# Autodesk Inventor assembly: robot
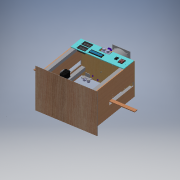
[picture p0: Inventor's stored thumbnail of the model, 180x180]
Saved by Autodesk Inventor 2017 (Build 210142000, 142)
## iProperties
Created: 2018-04-01
Part Number: robot
Document SubType Name: Assembly
Designer: franc
Mass: 1235.72 g
Surface Area: 6399.52 cm^2
Volume: 1204.8 cm^3
Density: 1.02566 g/cm^3
Author: franc
## Documents named in this file (16)
- C:\Users\franc\Desktop\EsialRobotik\Mecanique\2018\robot\robot.iam
- C:\Users\franc\Desktop\EsialRobotik\Mecanique\base_roulante\baseRoulante.iam
- C:\Users\franc\Desktop\EsialRobotik\Mecanique\2018\robot\socle-robot.ipt
- C:\Users\franc\Desktop\EsialRobotik\Mecanique\2018\robot\profile_alu.ipt
- C:\Users\franc\Desktop\EsialRobotik\Mecanique\2018\robot\abeille\lanceur-abeille.iam
- C:\Users\franc\Desktop\EsialRobotik\Mecanique\2018\robot\face-lateral.ipt
- C:\Users\franc\Desktop\EsialRobotik\Mecanique\2018\robot\abeille\lanceur-abeille 2.iam
- C:\Users\franc\Desktop\EsialRobotik\Mecanique\2018\robot\support_arriere.iam
- C:\Users\franc\Desktop\EsialRobotik\Mecanique\2018\robot\toit.ipt
- C:\Users\franc\Desktop\EsialRobotik\Mecanique\composants\SRF04\SRF04_sur_support.iam
- C:\Users\franc\Desktop\EsialRobotik\Mecanique\composants\Interrupteur\arret-urgence.ipt
- C:\Users\franc\Desktop\EsialRobotik\Mecanique\composants\RPlidar-A2M4\RPLIDAR A2.iam
- C:\Users\franc\Desktop\EsialRobotik\Mecanique\composants\Balises\support-balise.ipt
- C:\Users\franc\Desktop\EsialRobotik\Mecanique\composants\Balises\support-lidar.ipt
- C:\Users\franc\Desktop\EsialRobotik\Mecanique\composants\Balises\tige-filletee.ipt
- C:\Users\franc\Desktop\EsialRobotik\Mecanique\composants\Balises\cylindre-mat.ipt
## Components (26 placed, 15 different names)
1. baseRoulante:1 [sub-assembly] — Affleurement:1, Affleurement:2, Placage:1, Affleurement:6, Affleurement:7, Affleurement:9, Placage:29, Affleurement:10, Affleurement:12, Placage:32, Placage:34, Placage:66, Affleurement:31, Affleurement:32
2. socle-robot:1 — Affleurement:1, Affleurement:2, Placage:1, Placage:27, Affleurement:5, Affleurement:8, Placage:28, Placage:30, Affleurement:11, Placage:31, Placage:33, Affleurement:13, Placage:35, Placage:37, Affleurement:15, Placage:39
3. support_arriere:1 [sub-assembly] — Placage:43, Affleurement:16, Affleurement:17
4. arret-urgence:1 — Placage:53
5. SRF04_sur_support:1 [sub-assembly] — Placage:48, Affleurement:23, Placage:49
6. SRF04_sur_support:2 [sub-assembly] — Placage:45, Affleurement:20, Placage:52
7. SRF04_sur_support:3 [sub-assembly] — Placage:46, Affleurement:21, Placage:51
8. SRF04_sur_support:4 [sub-assembly] — Placage:47, Affleurement:22, Placage:50
9. toit:1 — Placage:44, Affleurement:18, Affleurement:19, Placage:45, Placage:46, Placage:47, Affleurement:20, Affleurement:21, Affleurement:22, Placage:48, Affleurement:23, Placage:49, Placage:50, Placage:51, Placage:52, Placage:53, Affleurement:24, Affleurement:25
10. lanceur-abeille 2:1 [sub-assembly] — Placage:40, Placage:41, Placage:42
11. lanceur-abeille:1 [sub-assembly] — Placage:36, Placage:37, Affleurement:14
12. profile_alu:1 — Affleurement:7, Affleurement:8, Placage:28, Placage:43
13. profile_alu:2 — Affleurement:9, Placage:29, Placage:30, Placage:38
14. profile_alu:3 — Affleurement:12, Placage:32, Placage:33
15. profile_alu:4 — Affleurement:10, Affleurement:11, Placage:31, Affleurement:17
16. face-lateral:1 — Placage:34, Affleurement:13, Placage:35, Placage:36, Affleurement:14, Affleurement:16, Placage:44, Affleurement:18, Affleurement:19
17. face-lateral:2 — Placage:38, Affleurement:15, Placage:39, Placage:40, Placage:41, Placage:42
18. cylindre-mat:1 — Placage:68, Tangente:1, Tangente:2
19. RPLIDAR A2:1 [sub-assembly] — Placage:54, Placage:55, Placage:56
20. support-balise:1 — Placage:61, Placage:62, Placage:63, Placage:68, Tangente:1, Tangente:2
21. support-lidar:1 — Placage:54, Placage:55, Placage:56, Placage:57, Placage:58, Placage:59, Placage:60, Placage:61, Placage:66, Affleurement:30, Placage:67
22. tige-filletee:1 — Placage:60, Placage:62, Affleurement:28
23. tige-filletee:2 — Placage:59, Affleurement:26, Placage:64
24. tige-filletee:3 — Placage:58, Placage:63, Affleurement:29
25. tige-filletee:4 — Placage:57, Placage:65, Affleurement:27
26. support-balise:2 — Affleurement:26, Placage:64, Placage:65, Affleurement:27, Affleurement:28, Affleurement:29, Affleurement:31
## Relationships (75: Mate 43, Flush 30, Tangent 2)
- Affleurement:1 [Flush] (5 mm): baseRoulante:1 ↔ socle-robot:1
- Affleurement:2 [Flush] (54 mm): baseRoulante:1 ↔ socle-robot:1
- Placage:1 [Mate]: baseRoulante:1 ↔ socle-robot:1
- Placage:27 [Mate]: socle-robot:1
- Affleurement:5 [Flush]: socle-robot:1
- Affleurement:6 [Flush] (340 mm): baseRoulante:1
- Affleurement:7 [Flush]: baseRoulante:1 ↔ profile_alu:1
- Affleurement:8 [Flush]: socle-robot:1 ↔ profile_alu:1
- Placage:28 [Mate]: socle-robot:1 ↔ profile_alu:1
- Affleurement:9 [Flush]: baseRoulante:1 ↔ profile_alu:2
- Placage:29 [Mate]: baseRoulante:1 ↔ profile_alu:2
- Placage:30 [Mate]: socle-robot:1 ↔ profile_alu:2
- Affleurement:10 [Flush]: baseRoulante:1 ↔ profile_alu:4
- Affleurement:11 [Flush]: socle-robot:1 ↔ profile_alu:4
- Placage:31 [Mate]: socle-robot:1 ↔ profile_alu:4
- Affleurement:12 [Flush]: baseRoulante:1 ↔ profile_alu:3
- Placage:32 [Mate]: baseRoulante:1 ↔ profile_alu:3
- Placage:33 [Mate]: socle-robot:1 ↔ profile_alu:3
- Placage:34 [Mate]: baseRoulante:1 ↔ face-lateral:1
- Affleurement:13 [Flush]: socle-robot:1 ↔ face-lateral:1
- Placage:35 [Mate]: socle-robot:1 ↔ face-lateral:1
- Placage:36 [Mate]: lanceur-abeille:1 ↔ face-lateral:1
- Placage:37 [Mate] (130 mm): socle-robot:1 ↔ lanceur-abeille:1
- Affleurement:14 [Flush] (81 mm): lanceur-abeille:1 ↔ face-lateral:1
- Placage:38 [Mate]: profile_alu:2 ↔ face-lateral:2
- Affleurement:15 [Flush]: socle-robot:1 ↔ face-lateral:2
- Placage:39 [Mate]: socle-robot:1 ↔ face-lateral:2
- Placage:40 [Mate]: lanceur-abeille 2:1 ↔ face-lateral:2
- Placage:41 [Mate]: lanceur-abeille 2:1 ↔ face-lateral:2
- Placage:42 [Mate]: lanceur-abeille 2:1 ↔ face-lateral:2
- Placage:43 [Mate]: support_arriere:1 ↔ profile_alu:1
- Affleurement:16 [Flush]: support_arriere:1 ↔ face-lateral:1
- Affleurement:17 [Flush]: support_arriere:1 ↔ profile_alu:4
- Placage:44 [Mate]: toit:1 ↔ face-lateral:1
- Affleurement:18 [Flush]: toit:1 ↔ face-lateral:1
- Affleurement:19 [Flush]: toit:1 ↔ face-lateral:1
- Placage:45 [Mate]: SRF04_sur_support:2 ↔ toit:1
- Placage:46 [Mate]: SRF04_sur_support:3 ↔ toit:1
- Placage:47 [Mate]: SRF04_sur_support:4 ↔ toit:1
- Affleurement:20 [Flush]: SRF04_sur_support:2 ↔ toit:1
- Affleurement:21 [Flush]: SRF04_sur_support:3 ↔ toit:1
- Affleurement:22 [Flush]: SRF04_sur_support:4 ↔ toit:1
- Placage:48 [Mate]: SRF04_sur_support:1 ↔ toit:1
- Affleurement:23 [Flush]: SRF04_sur_support:1 ↔ toit:1
- Placage:49 [Mate]: SRF04_sur_support:1 ↔ toit:1
- Placage:50 [Mate]: SRF04_sur_support:4 ↔ toit:1
- Placage:51 [Mate]: SRF04_sur_support:3 ↔ toit:1
- Placage:52 [Mate]: SRF04_sur_support:2 ↔ toit:1
- Placage:53 [Mate]: arret-urgence:1 ↔ toit:1
- Affleurement:24 [Flush] (-150 mm): toit:1
- Affleurement:25 [Flush] (-100 mm): toit:1
- Placage:54 [Mate]: RPLIDAR A2:1 ↔ support-lidar:1
- Placage:55 [Mate]: RPLIDAR A2:1 ↔ support-lidar:1
- Placage:56 [Mate]: RPLIDAR A2:1 ↔ support-lidar:1
- Placage:57 [Mate]: support-lidar:1 ↔ tige-filletee:4
- Placage:58 [Mate]: support-lidar:1 ↔ tige-filletee:3
- Placage:59 [Mate]: support-lidar:1 ↔ tige-filletee:2
- Placage:60 [Mate]: support-lidar:1 ↔ tige-filletee:1
- Placage:61 [Mate] (45 mm): support-balise:1 ↔ support-lidar:1
- Placage:62 [Mate]: support-balise:1 ↔ tige-filletee:1
- Placage:63 [Mate]: support-balise:1 ↔ tige-filletee:3
- Affleurement:26 [Flush]: tige-filletee:2 ↔ support-balise:2
- Placage:64 [Mate]: tige-filletee:2 ↔ support-balise:2
- Placage:65 [Mate]: tige-filletee:4 ↔ support-balise:2
- Affleurement:27 [Flush]: tige-filletee:4 ↔ support-balise:2
- Affleurement:28 [Flush]: tige-filletee:1 ↔ support-balise:2
- Affleurement:29 [Flush]: tige-filletee:3 ↔ support-balise:2
- Placage:66 [Mate] (330 mm): baseRoulante:1 ↔ support-lidar:1
- Affleurement:30 [Flush]: support-lidar:1
- Placage:67 [Mate]: support-lidar:1
- Affleurement:31 [Flush] (-430 mm): baseRoulante:1 ↔ support-balise:2
- Affleurement:32 [Flush] (350 mm): baseRoulante:1
- Placage:68 [Mate]: cylindre-mat:1 ↔ support-balise:1
- Tangente:1: cylindre-mat:1 ↔ support-balise:1
- Tangente:2: cylindre-mat:1 ↔ support-balise:1
